# Autodesk Inventor assembly: Piston5inch_v2
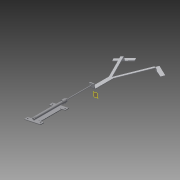
[picture p0: Inventor's stored thumbnail of the model, 180x180]
Saved by Autodesk Inventor 2013 (Build 170138000, 138)
## iProperties
Created: 2013-01-21
Part Number: Piston5inch_v2
Document SubType Name: Assembly
Designer: motoennies
Author: motoennies
## Documents named in this file (4)
- E:\Robotics\Hopper\Piston5inch_v2.iam
- \\NNHSSRV2.hs.sd203.org\MOToennies$\Inventor\Part10.ipt
- E:\Robotics\Hopper\Pneumatic Piston Bracket_v1.ipt
- E:\Robotics\Hopper\Feeder-Grabber_v2.ipt
## Components (3 placed, 3 different names)
1. Part10:1 — Mate:1, Angle:1, Flush:1, Mate:5
2. Pneumatic Piston Bracket_v1:1 — Mate:1, Angle:1, Flush:1, Mate:5, Mate:6, Mate:7, Flush:2
3. Feeder-Grabber_v2:1 — Mate:6, Mate:7, Flush:2
## Relationships (7: Mate 4, Flush 2, Angle 1)
- Mate:1 (10.16 mm): Part10:1 ↔ Pneumatic Piston Bracket_v1:1
- Angle:1 (180 deg): Part10:1 ↔ Pneumatic Piston Bracket_v1:1
- Flush:1 (5.08 mm): Part10:1 ↔ Pneumatic Piston Bracket_v1:1
- Mate:5 (-25.4 mm): Part10:1 ↔ Pneumatic Piston Bracket_v1:1
- Mate:6 (165.1 mm): Pneumatic Piston Bracket_v1:1 ↔ Feeder-Grabber_v2:1
- Mate:7 (-0.508 mm): Pneumatic Piston Bracket_v1:1 ↔ Feeder-Grabber_v2:1
- Flush:2 (9.2075 mm): Pneumatic Piston Bracket_v1:1 ↔ Feeder-Grabber_v2:1
